# Autodesk Inventor assembly: mirror_assembly_final
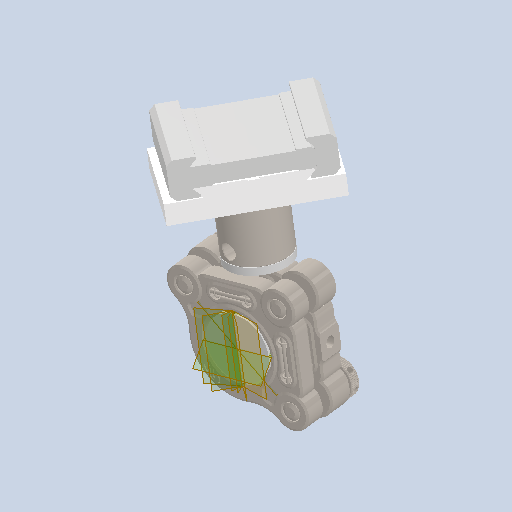
[picture p0: Inventor's stored thumbnail of the model, 512x512]
Saved by Autodesk Inventor 2026.1 (Build 301233000, 233)
## iProperties
Created: 2019-05-24
Part Number: mirror_assembly_final
Document SubType Name: Assembly
Designer: Julian
Author: Julian
## Documents named in this file (6)
- C:\Users\user\Desktop\setup for publishing\mirror_assembly_final - Kopie (2).iam
- C:\Users\user\Desktop\setup for publishing\XT66C2-Step_rail mount.ipt
- C:\Users\user\Desktop\setup for publishing\XT66D2-40-Step_post_mount.ipt
- C:\Users\user\Desktop\setup for publishing\SS100-F2H_suprema_1in_mirror_mount.ipt
- C:\Users\user\Desktop\setup for publishing\1in_5mm_mir.ipt
- C:\Users\user\Desktop\setup for publishing\PLS-P246_24,6_1in_PolarisPost + 3mm.ipt
## Components (5 placed, 5 different names)
1. XT66C2-Step_rail mount:1 — Passend:5, Passend:6, Fluchtend:1
2. XT66D2-40-Step_post_mount:1 — Passend:5, Passend:6, Fluchtend:1, Winkel:1, Winkel:2, Passend:9, Passend:10
3. SS100-F2H_suprema_1in_mirror_mount:1 — Passend:7, Passend:8, Passend:11, Passend:12
4. 1in_5mm_mir:1 — Passend:7, Passend:8, Winkel:1, Winkel:2
5. PLS-P246_24,6_1in_PolarisPost + 3mm:1 — Passend:9, Passend:10, Passend:11, Passend:12
## Relationships (11: Mate 8, Angle 2, Flush 1)
- Passend:5 [Mate]: XT66C2-Step_rail mount:1 ↔ XT66D2-40-Step_post_mount:1
- Passend:6 [Mate]: XT66C2-Step_rail mount:1 ↔ XT66D2-40-Step_post_mount:1
- Fluchtend:1 [Flush] (-0.0508 mm): XT66C2-Step_rail mount:1 ↔ XT66D2-40-Step_post_mount:1
- Passend:7 [Mate]: SS100-F2H_suprema_1in_mirror_mount:1 ↔ 1in_5mm_mir:1
- Passend:8 [Mate]: SS100-F2H_suprema_1in_mirror_mount:1 ↔ 1in_5mm_mir:1
- Winkel:1 [Angle] (45 deg): XT66D2-40-Step_post_mount:1 ↔ 1in_5mm_mir:1
- Winkel:2 [Angle] (0 deg): XT66D2-40-Step_post_mount:1 ↔ 1in_5mm_mir:1
- Passend:9 [Mate]: XT66D2-40-Step_post_mount:1 ↔ PLS-P246_24,6_1in_PolarisPost + 3mm:1
- Passend:10 [Mate]: XT66D2-40-Step_post_mount:1 ↔ PLS-P246_24,6_1in_PolarisPost + 3mm:1
- Passend:11 [Mate]: SS100-F2H_suprema_1in_mirror_mount:1 ↔ PLS-P246_24,6_1in_PolarisPost + 3mm:1
- Passend:12 [Mate]: SS100-F2H_suprema_1in_mirror_mount:1 ↔ PLS-P246_24,6_1in_PolarisPost + 3mm:1
